# Autodesk Inventor assembly: general
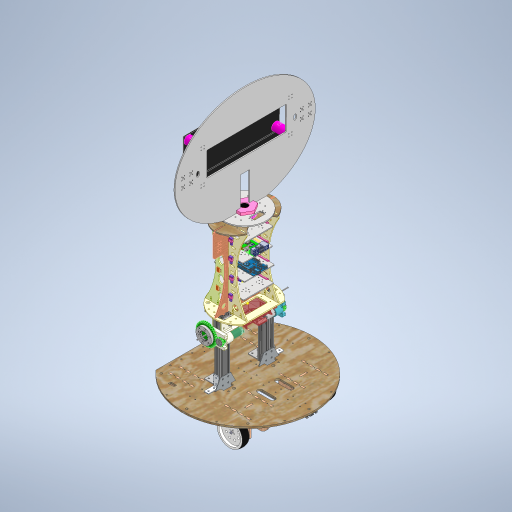
[picture p0: Inventor's stored thumbnail of the model, 512x512]
Saved by Autodesk Inventor 2024 (Build 280153000, 153)
## iProperties
Created: 2024-12-19
Part Number: general
Document SubType Name: Assembly
Designer: DELL
Author: DELL
## Documents named in this file (4)
- C:\Users\ejenie\reposGits\Cheburashka\Cheburashka_construction\general.iam
- C:\Users\ejenie\reposGits\Cheburashka\Cheburashka_construction\platform\platform.iam
- C:\Users\ejenie\reposGits\Cheburashka\Cheburashka_construction\korpus\korp.iam
- C:\Users\ejenie\reposGits\Cheburashka\Cheburashka_construction\face\лицо\Сборка1.iam
## Components (3 placed, 3 different names)
1. platform:1 [sub-assembly] — Заподлицо:1
2. korp:1 [sub-assembly] — Заподлицо:1, Совмещение:15, Совмещение:16, Совмещение:17
3. face [sub-assembly] — Совмещение:15, Совмещение:16, Совмещение:17
## Relationships (4: Mate 3, Flush 1)
- Заподлицо:1 [Flush]: platform:1 ↔ korp:1
- Совмещение:15 [Mate]: korp:1 ↔ face
- Совмещение:16 [Mate]: korp:1 ↔ face
- Совмещение:17 [Mate]: korp:1 ↔ face
